# Autodesk Inventor assembly: Motor Assembly
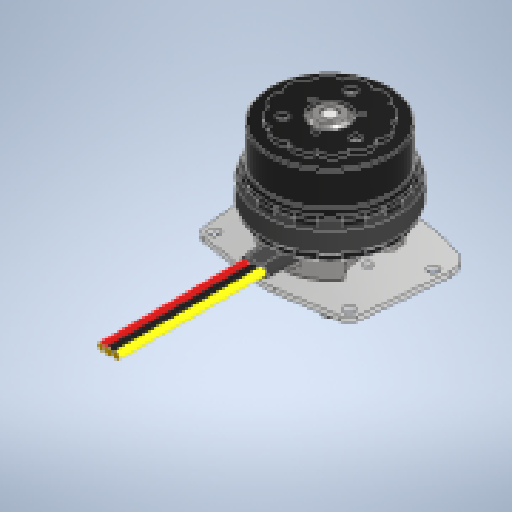
[picture p0: Inventor's stored thumbnail of the model, 512x512]
Saved by Autodesk Inventor 2023.2 (Build 272271000, 271)
## iProperties
Created: 2022-12-29
Part Number: Motor Assembly
Document SubType Name: Assembly
Designer: Nathan Cai
Mass: 100.216 g
Surface Area: 302.4 cm^2
Volume: 31.1645 cm^3
Density: 3.2157 g/cm^3
Author: Nathan Cai
## Documents named in this file (6)
- C:\Users\Nathan Cai\Documents\Inventor\Moon Cake V0.15\Motor Assembly.iam
- C:\Users\Nathan Cai\Documents\Inventor\Moon Cake V0.15\Motor Cap.ipt
- C:\Users\Nathan Cai\Documents\Inventor\Moon Cake V0.15\Motor Hub.ipt
- C:\Users\Nathan Cai\Documents\Inventor\Moon Cake V0.15\Motor Clutch.ipt
- C:\Users\Nathan Cai\Documents\Inventor\Moon Cake V0.15\Motor Plate.ipt
- C:\Users\Nathan Cai\Documents\Inventor\Moon Cake V0.15\Propdrive V2 3536D 1400KV\Propdrive V2 3536D 1400KV.iam
## Components (5 placed, 5 different names)
1. Motor Cap:1 — Mate:16, Mate:17, Mate:18
2. Motor Hub:1 — Mate:5, Mate:6, Mate:14, Mate:15
3. Motor Clutch:1 — Mate:5, Mate:6, Mate:13
4. Motor Plate:1 — Mate:9, Mate:11, Mate:12, Mate:13
5. Propdrive V2 3536D 1400KV:1 [sub-assembly] — Mate:9, Mate:11, Mate:12, Mate:14, Mate:15, Mate:16, Mate:17, Mate:18
## Relationships (11: Mate 11)
- Mate:5: Motor Hub:1 ↔ Motor Clutch:1
- Mate:6: Motor Hub:1 ↔ Motor Clutch:1
- Mate:9: Motor Plate:1 ↔ Propdrive V2 3536D 1400KV:1
- Mate:11: Motor Plate:1 ↔ Propdrive V2 3536D 1400KV:1
- Mate:12: Motor Plate:1 ↔ Propdrive V2 3536D 1400KV:1
- Mate:13 (11.1125 mm): Motor Clutch:1 ↔ Motor Plate:1
- Mate:14: Motor Hub:1 ↔ Propdrive V2 3536D 1400KV:1
- Mate:15: Motor Hub:1 ↔ Propdrive V2 3536D 1400KV:1
- Mate:16: Motor Cap:1 ↔ Propdrive V2 3536D 1400KV:1
- Mate:17: Motor Cap:1 ↔ Propdrive V2 3536D 1400KV:1
- Mate:18: Motor Cap:1 ↔ Propdrive V2 3536D 1400KV:1
